# Autodesk Inventor assembly: roue
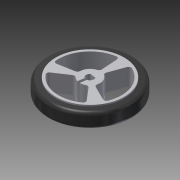
[picture p0: Inventor's stored thumbnail of the model, 180x180]
Saved by Autodesk Inventor 2014 SP2 (Build 180246200, 246)
## iProperties
Created: 2015-03-17
Part Number: roue
Document SubType Name: Assembly
Designer: sd
Mass: 2.78412 g
Surface Area: 33.231 cm^2
Volume: 2.80339 cm^3
Density: 0.993124 g/cm^3
Author: sd
## Documents named in this file (3)
- D:\Utilisateurs\sd\Mes documents\SVN\projets-gei\Dumber 2015\Mecanique\roue.iam
- D:\Utilisateurs\sd\Mes documents\SVN\projets-gei\Dumber 2015\Mecanique\Pneu.ipt
- D:\Utilisateurs\sd\Mes documents\SVN\projets-gei\Dumber 2015\Mecanique\Roue.ipt
## Components (2 placed, 2 different names)
1. Pneu:1 — Logement:1
2. Roue:1 — Logement:1
## Relationships (1: Insert 1)
- Logement:1 [Insert] (-0.5 mm): Pneu:1 ↔ Roue:1
